# Autodesk Inventor assembly: eMachineShop.20
(part 2 of 2)
- D:\Tesis\Modelo 3D\CAD\Electronicos\MC15A_V5\MC15A_V5_1779569544.214\MC15A_V5_1779569544.214\eMachineShop.20.315.ipt
- D:\Tesis\Modelo 3D\CAD\Electronicos\MC15A_V5\MC15A_V5_1779569544.214\MC15A_V5_1779569544.214\eMachineShop.20.316.ipt
- D:\Tesis\Modelo 3D\CAD\Electronicos\MC15A_V5\MC15A_V5_1779569544.214\MC15A_V5_1779569544.214\eMachineShop.20.317.ipt
- D:\Tesis\Modelo 3D\CAD\Electronicos\MC15A_V5\MC15A_V5_1779569544.214\MC15A_V5_1779569544.214\eMachineShop.20.318.ipt
- D:\Tesis\Modelo 3D\CAD\Electronicos\MC15A_V5\MC15A_V5_1779569544.214\MC15A_V5_1779569544.214\eMachineShop.20.319.ipt
- D:\Tesis\Modelo 3D\CAD\Electronicos\MC15A_V5\MC15A_V5_1779569544.214\MC15A_V5_1779569544.214\eMachineShop.20.320.ipt
- D:\Tesis\Modelo 3D\CAD\Electronicos\MC15A_V5\MC15A_V5_1779569544.214\MC15A_V5_1779569544.214\eMachineShop.20.321.ipt
- D:\Tesis\Modelo 3D\CAD\Electronicos\MC15A_V5\MC15A_V5_1779569544.214\MC15A_V5_1779569544.214\eMachineShop.20.322.ipt
- D:\Tesis\Modelo 3D\CAD\Electronicos\MC15A_V5\MC15A_V5_1779569544.214\MC15A_V5_1779569544.214\eMachineShop.20.323.ipt
- D:\Tesis\Modelo 3D\CAD\Electronicos\MC15A_V5\MC15A_V5_1779569544.214\MC15A_V5_1779569544.214\eMachineShop.20.324.ipt
- D:\Tesis\Modelo 3D\CAD\Electronicos\MC15A_V5\MC15A_V5_1779569544.214\MC15A_V5_1779569544.214\eMachineShop.20.325.ipt
- D:\Tesis\Modelo 3D\CAD\Electronicos\MC15A_V5\MC15A_V5_1779569544.214\MC15A_V5_1779569544.214\eMachineShop.20.326.ipt
- D:\Tesis\Modelo 3D\CAD\Electronicos\MC15A_V5\MC15A_V5_1779569544.214\MC15A_V5_1779569544.214\eMachineShop.20.327.ipt
- D:\Tesis\Modelo 3D\CAD\Electronicos\MC15A_V5\MC15A_V5_1779569544.214\MC15A_V5_1779569544.214\eMachineShop.20.328.ipt
- D:\Tesis\Modelo 3D\CAD\Electronicos\MC15A_V5\MC15A_V5_1779569544.214\MC15A_V5_1779569544.214\eMachineShop.20.329.ipt
- D:\Tesis\Modelo 3D\CAD\Electronicos\MC15A_V5\MC15A_V5_1779569544.214\MC15A_V5_1779569544.214\eMachineShop.20.330.ipt
- D:\Tesis\Modelo 3D\CAD\Electronicos\MC15A_V5\MC15A_V5_1779569544.214\MC15A_V5_1779569544.214\eMachineShop.20.331.ipt
- D:\Tesis\Modelo 3D\CAD\Electronicos\MC15A_V5\MC15A_V5_1779569544.214\MC15A_V5_1779569544.214\eMachineShop.20.332.ipt
- D:\Tesis\Modelo 3D\CAD\Electronicos\MC15A_V5\MC15A_V5_1779569544.214\MC15A_V5_1779569544.214\eMachineShop.20.333.ipt
- D:\Tesis\Modelo 3D\CAD\Electronicos\MC15A_V5\MC15A_V5_1779569544.214\MC15A_V5_1779569544.214\eMachineShop.20.334.ipt
- D:\Tesis\Modelo 3D\CAD\Electronicos\MC15A_V5\MC15A_V5_1779569544.214\MC15A_V5_1779569544.214\eMachineShop.20.335.ipt
- D:\Tesis\Modelo 3D\CAD\Electronicos\MC15A_V5\MC15A_V5_1779569544.214\MC15A_V5_1779569544.214\eMachineShop.20.336.ipt
- D:\Tesis\Modelo 3D\CAD\Electronicos\MC15A_V5\MC15A_V5_1779569544.214\MC15A_V5_1779569544.214\eMachineShop.20.337.ipt
- D:\Tesis\Modelo 3D\CAD\Electronicos\MC15A_V5\MC15A_V5_1779569544.214\MC15A_V5_1779569544.214\eMachineShop.20.338.ipt
- D:\Tesis\Modelo 3D\CAD\Electronicos\MC15A_V5\MC15A_V5_1779569544.214\MC15A_V5_1779569544.214\eMachineShop.20.339.ipt
- D:\Tesis\Modelo 3D\CAD\Electronicos\MC15A_V5\MC15A_V5_1779569544.214\MC15A_V5_1779569544.214\eMachineShop.20.340.ipt
- D:\Tesis\Modelo 3D\CAD\Electronicos\MC15A_V5\MC15A_V5_1779569544.214\MC15A_V5_1779569544.214\eMachineShop.20.341.ipt
- D:\Tesis\Modelo 3D\CAD\Electronicos\MC15A_V5\MC15A_V5_1779569544.214\MC15A_V5_1779569544.214\eMachineShop.20.342.ipt
- D:\Tesis\Modelo 3D\CAD\Electronicos\MC15A_V5\MC15A_V5_1779569544.214\MC15A_V5_1779569544.214\eMachineShop.20.343.ipt
- D:\Tesis\Modelo 3D\CAD\Electronicos\MC15A_V5\MC15A_V5_1779569544.214\MC15A_V5_1779569544.214\eMachineShop.20.344.ipt
- D:\Tesis\Modelo 3D\CAD\Electronicos\MC15A_V5\MC15A_V5_1779569544.214\MC15A_V5_1779569544.214\eMachineShop.20.345.ipt
- D:\Tesis\Modelo 3D\CAD\Electronicos\MC15A_V5\MC15A_V5_1779569544.214\MC15A_V5_1779569544.214\eMachineShop.20.346.ipt
- D:\Tesis\Modelo 3D\CAD\Electronicos\MC15A_V5\MC15A_V5_1779569544.214\MC15A_V5_1779569544.214\eMachineShop.20.347.ipt
- D:\Tesis\Modelo 3D\CAD\Electronicos\MC15A_V5\MC15A_V5_1779569544.214\MC15A_V5_1779569544.214\eMachineShop.20.348.ipt
- D:\Tesis\Modelo 3D\CAD\Electronicos\MC15A_V5\MC15A_V5_1779569544.214\MC15A_V5_1779569544.214\eMachineShop.20.349.ipt
- D:\Tesis\Modelo 3D\CAD\Electronicos\MC15A_V5\MC15A_V5_1779569544.214\MC15A_V5_1779569544.214\eMachineShop.20.350.ipt
- D:\Tesis\Modelo 3D\CAD\Electronicos\MC15A_V5\MC15A_V5_1779569544.214\MC15A_V5_1779569544.214\eMachineShop.20.351.ipt
- D:\Tesis\Modelo 3D\CAD\Electronicos\MC15A_V5\MC15A_V5_1779569544.214\MC15A_V5_1779569544.214\eMachineShop.20.352.ipt
- D:\Tesis\Modelo 3D\CAD\Electronicos\MC15A_V5\MC15A_V5_1779569544.214\MC15A_V5_1779569544.214\eMachineShop.20.353.ipt
- D:\Tesis\Modelo 3D\CAD\Electronicos\MC15A_V5\MC15A_V5_1779569544.214\MC15A_V5_1779569544.214\eMachineShop.20.354.ipt
- D:\Tesis\Modelo 3D\CAD\Electronicos\MC15A_V5\MC15A_V5_1779569544.214\MC15A_V5_1779569544.214\eMachineShop.20.355.ipt
- D:\Tesis\Modelo 3D\CAD\Electronicos\MC15A_V5\MC15A_V5_1779569544.214\MC15A_V5_1779569544.214\eMachineShop.20.356.ipt
- D:\Tesis\Modelo 3D\CAD\Electronicos\MC15A_V5\MC15A_V5_1779569544.214\MC15A_V5_1779569544.214\eMachineShop.20.357.ipt
- D:\Tesis\Modelo 3D\CAD\Electronicos\MC15A_V5\MC15A_V5_1779569544.214\MC15A_V5_1779569544.214\eMachineShop.20.358.ipt
- D:\Tesis\Modelo 3D\CAD\Electronicos\MC15A_V5\MC15A_V5_1779569544.214\MC15A_V5_1779569544.214\eMachineShop.20.359.ipt
- D:\Tesis\Modelo 3D\CAD\Electronicos\MC15A_V5\MC15A_V5_1779569544.214\MC15A_V5_1779569544.214\eMachineShop.20.360.ipt
- D:\Tesis\Modelo 3D\CAD\Electronicos\MC15A_V5\MC15A_V5_1779569544.214\MC15A_V5_1779569544.214\eMachineShop.20.361.ipt
- D:\Tesis\Modelo 3D\CAD\Electronicos\MC15A_V5\MC15A_V5_1779569544.214\MC15A_V5_1779569544.214\eMachineShop.20.362.ipt
- D:\Tesis\Modelo 3D\CAD\Electronicos\MC15A_V5\MC15A_V5_1779569544.214\MC15A_V5_1779569544.214\eMachineShop.20.363.ipt
- D:\Tesis\Modelo 3D\CAD\Electronicos\MC15A_V5\MC15A_V5_1779569544.214\MC15A_V5_1779569544.214\eMachineShop.20.364.ipt
- D:\Tesis\Modelo 3D\CAD\Electronicos\MC15A_V5\MC15A_V5_1779569544.214\MC15A_V5_1779569544.214\eMachineShop.20.365.ipt
- D:\Tesis\Modelo 3D\CAD\Electronicos\MC15A_V5\MC15A_V5_1779569544.214\MC15A_V5_1779569544.214\eMachineShop.20.366.ipt
- D:\Tesis\Modelo 3D\CAD\Electronicos\MC15A_V5\MC15A_V5_1779569544.214\MC15A_V5_1779569544.214\eMachineShop.20.367.ipt
- D:\Tesis\Modelo 3D\CAD\Electronicos\MC15A_V5\MC15A_V5_1779569544.214\MC15A_V5_1779569544.214\eMachineShop.20.368.ipt
- D:\Tesis\Modelo 3D\CAD\Electronicos\MC15A_V5\MC15A_V5_1779569544.214\MC15A_V5_1779569544.214\eMachineShop.20.369.ipt
- D:\Tesis\Modelo 3D\CAD\Electronicos\MC15A_V5\MC15A_V5_1779569544.214\MC15A_V5_1779569544.214\eMachineShop.20.370.ipt
- D:\Tesis\Modelo 3D\CAD\Electronicos\MC15A_V5\MC15A_V5_1779569544.214\MC15A_V5_1779569544.214\eMachineShop.20.371.ipt
- D:\Tesis\Modelo 3D\CAD\Electronicos\MC15A_V5\MC15A_V5_1779569544.214\MC15A_V5_1779569544.214\eMachineShop.20.372.ipt
- D:\Tesis\Modelo 3D\CAD\Electronicos\MC15A_V5\MC15A_V5_1779569544.214\MC15A_V5_1779569544.214\eMachineShop.20.373.ipt
- D:\Tesis\Modelo 3D\CAD\Electronicos\MC15A_V5\MC15A_V5_1779569544.214\MC15A_V5_1779569544.214\eMachineShop.20.374.ipt
- D:\Tesis\Modelo 3D\CAD\Electronicos\MC15A_V5\MC15A_V5_1779569544.214\MC15A_V5_1779569544.214\eMachineShop.20.375.ipt
- D:\Tesis\Modelo 3D\CAD\Electronicos\MC15A_V5\MC15A_V5_1779569544.214\MC15A_V5_1779569544.214\eMachineShop.20.376.ipt
- D:\Tesis\Modelo 3D\CAD\Electronicos\MC15A_V5\MC15A_V5_1779569544.214\MC15A_V5_1779569544.214\eMachineShop.20.377.ipt
- D:\Tesis\Modelo 3D\CAD\Electronicos\MC15A_V5\MC15A_V5_1779569544.214\MC15A_V5_1779569544.214\eMachineShop.20.378.ipt
- D:\Tesis\Modelo 3D\CAD\Electronicos\MC15A_V5\MC15A_V5_1779569544.214\MC15A_V5_1779569544.214\eMachineShop.20.379.ipt
- D:\Tesis\Modelo 3D\CAD\Electronicos\MC15A_V5\MC15A_V5_1779569544.214\MC15A_V5_1779569544.214\eMachineShop.20.380.ipt
- D:\Tesis\Modelo 3D\CAD\Electronicos\MC15A_V5\MC15A_V5_1779569544.214\MC15A_V5_1779569544.214\eMachineShop.20.381.ipt
- D:\Tesis\Modelo 3D\CAD\Electronicos\MC15A_V5\MC15A_V5_1779569544.214\MC15A_V5_1779569544.214\eMachineShop.20.382.ipt
- D:\Tesis\Modelo 3D\CAD\Electronicos\MC15A_V5\MC15A_V5_1779569544.214\MC15A_V5_1779569544.214\eMachineShop.20.383.ipt
- D:\Tesis\Modelo 3D\CAD\Electronicos\MC15A_V5\MC15A_V5_1779569544.214\MC15A_V5_1779569544.214\eMachineShop.20.384.ipt
- D:\Tesis\Modelo 3D\CAD\Electronicos\MC15A_V5\MC15A_V5_1779569544.214\MC15A_V5_1779569544.214\eMachineShop.20.385.ipt
- D:\Tesis\Modelo 3D\CAD\Electronicos\MC15A_V5\MC15A_V5_1779569544.214\MC15A_V5_1779569544.214\eMachineShop.20.386.ipt
- D:\Tesis\Modelo 3D\CAD\Electronicos\MC15A_V5\MC15A_V5_1779569544.214\MC15A_V5_1779569544.214\eMachineShop.20.387.ipt
- D:\Tesis\Modelo 3D\CAD\Electronicos\MC15A_V5\MC15A_V5_1779569544.214\MC15A_V5_1779569544.214\eMachineShop.20.388.ipt
- D:\Tesis\Modelo 3D\CAD\Electronicos\MC15A_V5\MC15A_V5_1779569544.214\MC15A_V5_1779569544.214\eMachineShop.20.389.ipt
- D:\Tesis\Modelo 3D\CAD\Electronicos\MC15A_V5\MC15A_V5_1779569544.214\MC15A_V5_1779569544.214\eMachineShop.20.390.ipt
- D:\Tesis\Modelo 3D\CAD\Electronicos\MC15A_V5\MC15A_V5_1779569544.214\MC15A_V5_1779569544.214\eMachineShop.20.391.ipt
- D:\Tesis\Modelo 3D\CAD\Electronicos\MC15A_V5\MC15A_V5_1779569544.214\MC15A_V5_1779569544.214\eMachineShop.20.392.ipt
- D:\Tesis\Modelo 3D\CAD\Electronicos\MC15A_V5\MC15A_V5_1779569544.214\MC15A_V5_1779569544.214\eMachineShop.20.393.ipt
- D:\Tesis\Modelo 3D\CAD\Electronicos\MC15A_V5\MC15A_V5_1779569544.214\MC15A_V5_1779569544.214\eMachineShop.20.394.ipt
- D:\Tesis\Modelo 3D\CAD\Electronicos\MC15A_V5\MC15A_V5_1779569544.214\MC15A_V5_1779569544.214\eMachineShop.20.395.ipt
- D:\Tesis\Modelo 3D\CAD\Electronicos\MC15A_V5\MC15A_V5_1779569544.214\MC15A_V5_1779569544.214\eMachineShop.20.396.ipt
- D:\Tesis\Modelo 3D\CAD\Electronicos\MC15A_V5\MC15A_V5_1779569544.214\MC15A_V5_1779569544.214\eMachineShop.20.397.ipt
- D:\Tesis\Modelo 3D\CAD\Electronicos\MC15A_V5\MC15A_V5_1779569544.214\MC15A_V5_1779569544.214\eMachineShop.20.398.ipt
- D:\Tesis\Modelo 3D\CAD\Electronicos\MC15A_V5\MC15A_V5_1779569544.214\MC15A_V5_1779569544.214\eMachineShop.20.399.ipt
- D:\Tesis\Modelo 3D\CAD\Electronicos\MC15A_V5\MC15A_V5_1779569544.214\MC15A_V5_1779569544.214\eMachineShop.20.400.ipt
- D:\Tesis\Modelo 3D\CAD\Electronicos\MC15A_V5\MC15A_V5_1779569544.214\MC15A_V5_1779569544.214\eMachineShop.20.401.ipt
- D:\Tesis\Modelo 3D\CAD\Electronicos\MC15A_V5\MC15A_V5_1779569544.214\MC15A_V5_1779569544.214\eMachineShop.20.402.ipt
- D:\Tesis\Modelo 3D\CAD\Electronicos\MC15A_V5\MC15A_V5_1779569544.214\MC15A_V5_1779569544.214\eMachineShop.20.403.ipt
- D:\Tesis\Modelo 3D\CAD\Electronicos\MC15A_V5\MC15A_V5_1779569544.214\MC15A_V5_1779569544.214\eMachineShop.20.404.ipt
- D:\Tesis\Modelo 3D\CAD\Electronicos\MC15A_V5\MC15A_V5_1779569544.214\MC15A_V5_1779569544.214\eMachineShop.20.405.ipt
- D:\Tesis\Modelo 3D\CAD\Electronicos\MC15A_V5\MC15A_V5_1779569544.214\MC15A_V5_1779569544.214\eMachineShop.20.406.ipt
- D:\Tesis\Modelo 3D\CAD\Electronicos\MC15A_V5\MC15A_V5_1779569544.214\MC15A_V5_1779569544.214\eMachineShop.20.407.ipt
- D:\Tesis\Modelo 3D\CAD\Electronicos\MC15A_V5\MC15A_V5_1779569544.214\MC15A_V5_1779569544.214\eMachineShop.20.408.ipt
- D:\Tesis\Modelo 3D\CAD\Electronicos\MC15A_V5\MC15A_V5_1779569544.214\MC15A_V5_1779569544.214\eMachineShop.20.409.ipt
- D:\Tesis\Modelo 3D\CAD\Electronicos\MC15A_V5\MC15A_V5_1779569544.214\MC15A_V5_1779569544.214\eMachineShop.20.410.ipt
- D:\Tesis\Modelo 3D\CAD\Electronicos\MC15A_V5\MC15A_V5_1779569544.214\MC15A_V5_1779569544.214\eMachineShop.20.411.ipt
- D:\Tesis\Modelo 3D\CAD\Electronicos\MC15A_V5\MC15A_V5_1779569544.214\MC15A_V5_1779569544.214\eMachineShop.20.412.ipt
- D:\Tesis\Modelo 3D\CAD\Electronicos\MC15A_V5\MC15A_V5_1779569544.214\MC15A_V5_1779569544.214\eMachineShop.20.413.ipt
- D:\Tesis\Modelo 3D\CAD\Electronicos\MC15A_V5\MC15A_V5_1779569544.214\MC15A_V5_1779569544.214\eMachineShop.20.414.ipt
- D:\Tesis\Modelo 3D\CAD\Electronicos\MC15A_V5\MC15A_V5_1779569544.214\MC15A_V5_1779569544.214\eMachineShop.20.415.ipt
- D:\Tesis\Modelo 3D\CAD\Electronicos\MC15A_V5\MC15A_V5_1779569544.214\MC15A_V5_1779569544.214\eMachineShop.20.416.ipt
- D:\Tesis\Modelo 3D\CAD\Electronicos\MC15A_V5\MC15A_V5_1779569544.214\MC15A_V5_1779569544.214\eMachineShop.20.417.ipt
- D:\Tesis\Modelo 3D\CAD\Electronicos\MC15A_V5\MC15A_V5_1779569544.214\MC15A_V5_1779569544.214\eMachineShop.20.418.ipt
- D:\Tesis\Modelo 3D\CAD\Electronicos\MC15A_V5\MC15A_V5_1779569544.214\MC15A_V5_1779569544.214\eMachineShop.20.419.ipt
- D:\Tesis\Modelo 3D\CAD\Electronicos\MC15A_V5\MC15A_V5_1779569544.214\MC15A_V5_1779569544.214\eMachineShop.20.420.ipt
- D:\Tesis\Modelo 3D\CAD\Electronicos\MC15A_V5\MC15A_V5_1779569544.214\MC15A_V5_1779569544.214\eMachineShop.20.421.ipt
- D:\Tesis\Modelo 3D\CAD\Electronicos\MC15A_V5\MC15A_V5_1779569544.214\MC15A_V5_1779569544.214\eMachineShop.20.422.ipt
- D:\Tesis\Modelo 3D\CAD\Electronicos\MC15A_V5\MC15A_V5_1779569544.214\MC15A_V5_1779569544.214\eMachineShop.20.423.ipt
- D:\Tesis\Modelo 3D\CAD\Electronicos\MC15A_V5\MC15A_V5_1779569544.214\MC15A_V5_1779569544.214\eMachineShop.20.424.ipt
- D:\Tesis\Modelo 3D\CAD\Electronicos\MC15A_V5\MC15A_V5_1779569544.214\MC15A_V5_1779569544.214\eMachineShop.20.425.ipt
- D:\Tesis\Modelo 3D\CAD\Electronicos\MC15A_V5\MC15A_V5_1779569544.214\MC15A_V5_1779569544.214\eMachineShop.20.426.ipt
- D:\Tesis\Modelo 3D\CAD\Electronicos\MC15A_V5\MC15A_V5_1779569544.214\MC15A_V5_1779569544.214\eMachineShop.20.427.ipt
- D:\Tesis\Modelo 3D\CAD\Electronicos\MC15A_V5\MC15A_V5_1779569544.214\MC15A_V5_1779569544.214\eMachineShop.20.428.ipt
- D:\Tesis\Modelo 3D\CAD\Electronicos\MC15A_V5\MC15A_V5_1779569544.214\MC15A_V5_1779569544.214\eMachineShop.20.429.ipt
- D:\Tesis\Modelo 3D\CAD\Electronicos\MC15A_V5\MC15A_V5_1779569544.214\MC15A_V5_1779569544.214\eMachineShop.20.430.ipt
- D:\Tesis\Modelo 3D\CAD\Electronicos\MC15A_V5\MC15A_V5_1779569544.214\MC15A_V5_1779569544.214\eMachineShop.20.431.ipt
- D:\Tesis\Modelo 3D\CAD\Electronicos\MC15A_V5\MC15A_V5_1779569544.214\MC15A_V5_1779569544.214\eMachineShop.20.432.ipt
- D:\Tesis\Modelo 3D\CAD\Electronicos\MC15A_V5\MC15A_V5_1779569544.214\MC15A_V5_1779569544.214\eMachineShop.20.433.ipt
- D:\Tesis\Modelo 3D\CAD\Electronicos\MC15A_V5\MC15A_V5_1779569544.214\MC15A_V5_1779569544.214\eMachineShop.20.434.ipt
- D:\Tesis\Modelo 3D\CAD\Electronicos\MC15A_V5\MC15A_V5_1779569544.214\MC15A_V5_1779569544.214\eMachineShop.20.435.ipt
- D:\Tesis\Modelo 3D\CAD\Electronicos\MC15A_V5\MC15A_V5_1779569544.214\MC15A_V5_1779569544.214\eMachineShop.20.436.ipt
- D:\Tesis\Modelo 3D\CAD\Electronicos\MC15A_V5\MC15A_V5_1779569544.214\MC15A_V5_1779569544.214\eMachineShop.20.437.ipt
- D:\Tesis\Modelo 3D\CAD\Electronicos\MC15A_V5\MC15A_V5_1779569544.214\MC15A_V5_1779569544.214\eMachineShop.20.438.ipt
- D:\Tesis\Modelo 3D\CAD\Electronicos\MC15A_V5\MC15A_V5_1779569544.214\MC15A_V5_1779569544.214\eMachineShop.20.439.ipt
- D:\Tesis\Modelo 3D\CAD\Electronicos\MC15A_V5\MC15A_V5_1779569544.214\MC15A_V5_1779569544.214\eMachineShop.20.440.ipt
- D:\Tesis\Modelo 3D\CAD\Electronicos\MC15A_V5\MC15A_V5_1779569544.214\MC15A_V5_1779569544.214\eMachineShop.20.441.ipt
- D:\Tesis\Modelo 3D\CAD\Electronicos\MC15A_V5\MC15A_V5_1779569544.214\MC15A_V5_1779569544.214\eMachineShop.20.442.ipt
- D:\Tesis\Modelo 3D\CAD\Electronicos\MC15A_V5\MC15A_V5_1779569544.214\MC15A_V5_1779569544.214\eMachineShop.20.443.ipt
- D:\Tesis\Modelo 3D\CAD\Electronicos\MC15A_V5\MC15A_V5_1779569544.214\MC15A_V5_1779569544.214\eMachineShop.20.444.ipt
- D:\Tesis\Modelo 3D\CAD\Electronicos\MC15A_V5\MC15A_V5_1779569544.214\MC15A_V5_1779569544.214\eMachineShop.20.445.ipt
- D:\Tesis\Modelo 3D\CAD\Electronicos\MC15A_V5\MC15A_V5_1779569544.214\MC15A_V5_1779569544.214\eMachineShop.20.446.ipt
- D:\Tesis\Modelo 3D\CAD\Electronicos\MC15A_V5\MC15A_V5_1779569544.214\MC15A_V5_1779569544.214\eMachineShop.20.447.ipt
- D:\Tesis\Modelo 3D\CAD\Electronicos\MC15A_V5\MC15A_V5_1779569544.214\MC15A_V5_1779569544.214\eMachineShop.20.448.ipt
- D:\Tesis\Modelo 3D\CAD\Electronicos\MC15A_V5\MC15A_V5_1779569544.214\MC15A_V5_1779569544.214\eMachineShop.20.449.ipt
- D:\Tesis\Modelo 3D\CAD\Electronicos\MC15A_V5\MC15A_V5_1779569544.214\MC15A_V5_1779569544.214\eMachineShop.20.450.ipt
- D:\Tesis\Modelo 3D\CAD\Electronicos\MC15A_V5\MC15A_V5_1779569544.214\MC15A_V5_1779569544.214\eMachineShop.20.451.ipt
- D:\Tesis\Modelo 3D\CAD\Electronicos\MC15A_V5\MC15A_V5_1779569544.214\MC15A_V5_1779569544.214\eMachineShop.20.452.ipt
- D:\Tesis\Modelo 3D\CAD\Electronicos\MC15A_V5\MC15A_V5_1779569544.214\MC15A_V5_1779569544.214\eMachineShop.20.453.ipt
- D:\Tesis\Modelo 3D\CAD\Electronicos\MC15A_V5\MC15A_V5_1779569544.214\MC15A_V5_1779569544.214\eMachineShop.20.454.ipt
- D:\Tesis\Modelo 3D\CAD\Electronicos\MC15A_V5\MC15A_V5_1779569544.214\MC15A_V5_1779569544.214\eMachineShop.20.455.ipt
- D:\Tesis\Modelo 3D\CAD\Electronicos\MC15A_V5\MC15A_V5_1779569544.214\MC15A_V5_1779569544.214\eMachineShop.20.456.ipt
- D:\Tesis\Modelo 3D\CAD\Electronicos\MC15A_V5\MC15A_V5_1779569544.214\MC15A_V5_1779569544.214\eMachineShop.20.457.ipt
- D:\Tesis\Modelo 3D\CAD\Electronicos\MC15A_V5\MC15A_V5_1779569544.214\MC15A_V5_1779569544.214\eMachineShop.20.458.ipt
- D:\Tesis\Modelo 3D\CAD\Electronicos\MC15A_V5\MC15A_V5_1779569544.214\MC15A_V5_1779569544.214\eMachineShop.20.459.ipt
- D:\Tesis\Modelo 3D\CAD\Electronicos\MC15A_V5\MC15A_V5_1779569544.214\MC15A_V5_1779569544.214\eMachineShop.20.460.ipt
- D:\Tesis\Modelo 3D\CAD\Electronicos\MC15A_V5\MC15A_V5_1779569544.214\MC15A_V5_1779569544.214\eMachineShop.20.461.ipt
- D:\Tesis\Modelo 3D\CAD\Electronicos\MC15A_V5\MC15A_V5_1779569544.214\MC15A_V5_1779569544.214\eMachineShop.20.462.ipt
- D:\Tesis\Modelo 3D\CAD\Electronicos\MC15A_V5\MC15A_V5_1779569544.214\MC15A_V5_1779569544.214\eMachineShop.20.463.ipt
- D:\Tesis\Modelo 3D\CAD\Electronicos\MC15A_V5\MC15A_V5_1779569544.214\MC15A_V5_1779569544.214\eMachineShop.20.464.ipt
- D:\Tesis\Modelo 3D\CAD\Electronicos\MC15A_V5\MC15A_V5_1779569544.214\MC15A_V5_1779569544.214\eMachineShop.20.465.ipt
- D:\Tesis\Modelo 3D\CAD\Electronicos\MC15A_V5\MC15A_V5_1779569544.214\MC15A_V5_1779569544.214\eMachineShop.20.466.ipt
- D:\Tesis\Modelo 3D\CAD\Electronicos\MC15A_V5\MC15A_V5_1779569544.214\MC15A_V5_1779569544.214\eMachineShop.20.467.ipt
- D:\Tesis\Modelo 3D\CAD\Electronicos\MC15A_V5\MC15A_V5_1779569544.214\MC15A_V5_1779569544.214\eMachineShop.20.468.ipt
- D:\Tesis\Modelo 3D\CAD\Electronicos\MC15A_V5\MC15A_V5_1779569544.214\MC15A_V5_1779569544.214\eMachineShop.20.469.ipt
- D:\Tesis\Modelo 3D\CAD\Electronicos\MC15A_V5\MC15A_V5_1779569544.214\MC15A_V5_1779569544.214\eMachineShop.20.470.ipt
- D:\Tesis\Modelo 3D\CAD\Electronicos\MC15A_V5\MC15A_V5_1779569544.214\MC15A_V5_1779569544.214\eMachineShop.20.471.ipt
- D:\Tesis\Modelo 3D\CAD\Electronicos\MC15A_V5\MC15A_V5_1779569544.214\MC15A_V5_1779569544.214\eMachineShop.20.472.ipt
- D:\Tesis\Modelo 3D\CAD\Electronicos\MC15A_V5\MC15A_V5_1779569544.214\MC15A_V5_1779569544.214\eMachineShop.20.473.ipt
- D:\Tesis\Modelo 3D\CAD\Electronicos\MC15A_V5\MC15A_V5_1779569544.214\MC15A_V5_1779569544.214\eMachineShop.20.474.ipt
- D:\Tesis\Modelo 3D\CAD\Electronicos\MC15A_V5\MC15A_V5_1779569544.214\MC15A_V5_1779569544.214\eMachineShop.20.475.ipt
- D:\Tesis\Modelo 3D\CAD\Electronicos\MC15A_V5\MC15A_V5_1779569544.214\MC15A_V5_1779569544.214\eMachineShop.20.476.ipt
- D:\Tesis\Modelo 3D\CAD\Electronicos\MC15A_V5\MC15A_V5_1779569544.214\MC15A_V5_1779569544.214\eMachineShop.20.477.ipt
- D:\Tesis\Modelo 3D\CAD\Electronicos\MC15A_V5\MC15A_V5_1779569544.214\MC15A_V5_1779569544.214\eMachineShop.20.478.ipt
- D:\Tesis\Modelo 3D\CAD\Electronicos\MC15A_V5\MC15A_V5_1779569544.214\MC15A_V5_1779569544.214\eMachineShop.20.479.ipt
- D:\Tesis\Modelo 3D\CAD\Electronicos\MC15A_V5\MC15A_V5_1779569544.214\MC15A_V5_1779569544.214\eMachineShop.20.480.ipt
- D:\Tesis\Modelo 3D\CAD\Electronicos\MC15A_V5\MC15A_V5_1779569544.214\MC15A_V5_1779569544.214\eMachineShop.20.481.ipt
- D:\Tesis\Modelo 3D\CAD\Electronicos\MC15A_V5\MC15A_V5_1779569544.214\MC15A_V5_1779569544.214\eMachineShop.20.482.ipt
- D:\Tesis\Modelo 3D\CAD\Electronicos\MC15A_V5\MC15A_V5_1779569544.214\MC15A_V5_1779569544.214\eMachineShop.20.483.ipt
- D:\Tesis\Modelo 3D\CAD\Electronicos\MC15A_V5\MC15A_V5_1779569544.214\MC15A_V5_1779569544.214\eMachineShop.20.484.ipt
- D:\Tesis\Modelo 3D\CAD\Electronicos\MC15A_V5\MC15A_V5_1779569544.214\MC15A_V5_1779569544.214\eMachineShop.20.485.ipt
- D:\Tesis\Modelo 3D\CAD\Electronicos\MC15A_V5\MC15A_V5_1779569544.214\MC15A_V5_1779569544.214\eMachineShop.20.486.ipt
- D:\Tesis\Modelo 3D\CAD\Electronicos\MC15A_V5\MC15A_V5_1779569544.214\MC15A_V5_1779569544.214\eMachineShop.20.487.ipt
- D:\Tesis\Modelo 3D\CAD\Electronicos\MC15A_V5\MC15A_V5_1779569544.214\MC15A_V5_1779569544.214\eMachineShop.20.488.ipt
- D:\Tesis\Modelo 3D\CAD\Electronicos\MC15A_V5\MC15A_V5_1779569544.214\MC15A_V5_1779569544.214\eMachineShop.20.489.ipt
- D:\Tesis\Modelo 3D\CAD\Electronicos\MC15A_V5\MC15A_V5_1779569544.214\MC15A_V5_1779569544.214\eMachineShop.20.490.ipt
- D:\Tesis\Modelo 3D\CAD\Electronicos\MC15A_V5\MC15A_V5_1779569544.214\MC15A_V5_1779569544.214\eMachineShop.20.491.ipt
- D:\Tesis\Modelo 3D\CAD\Electronicos\MC15A_V5\MC15A_V5_1779569544.214\MC15A_V5_1779569544.214\eMachineShop.20.492.ipt
- D:\Tesis\Modelo 3D\CAD\Electronicos\MC15A_V5\MC15A_V5_1779569544.214\MC15A_V5_1779569544.214\eMachineShop.20.493.ipt
- D:\Tesis\Modelo 3D\CAD\Electronicos\MC15A_V5\MC15A_V5_1779569544.214\MC15A_V5_1779569544.214\eMachineShop.20.494.ipt
- D:\Tesis\Modelo 3D\CAD\Electronicos\MC15A_V5\MC15A_V5_1779569544.214\MC15A_V5_1779569544.214\eMachineShop.20.495.ipt
- D:\Tesis\Modelo 3D\CAD\Electronicos\MC15A_V5\MC15A_V5_1779569544.214\MC15A_V5_1779569544.214\eMachineShop.20.496.ipt
- D:\Tesis\Modelo 3D\CAD\Electronicos\MC15A_V5\MC15A_V5_1779569544.214\MC15A_V5_1779569544.214\eMachineShop.20.497.ipt
- D:\Tesis\Modelo 3D\CAD\Electronicos\MC15A_V5\MC15A_V5_1779569544.214\MC15A_V5_1779569544.214\eMachineShop.20.498.ipt
- D:\Tesis\Modelo 3D\CAD\Electronicos\MC15A_V5\MC15A_V5_1779569544.214\MC15A_V5_1779569544.214\eMachineShop.20.499.ipt
- D:\Tesis\Modelo 3D\CAD\Electronicos\MC15A_V5\MC15A_V5_1779569544.214\MC15A_V5_1779569544.214\eMachineShop.20.500.ipt
- D:\Tesis\Modelo 3D\CAD\Electronicos\MC15A_V5\MC15A_V5_1779569544.214\MC15A_V5_1779569544.214\eMachineShop.20.501.ipt
- D:\Tesis\Modelo 3D\CAD\Electronicos\MC15A_V5\MC15A_V5_1779569544.214\MC15A_V5_1779569544.214\eMachineShop.20.502.ipt
- D:\Tesis\Modelo 3D\CAD\Electronicos\MC15A_V5\MC15A_V5_1779569544.214\MC15A_V5_1779569544.214\eMachineShop.20.503.ipt
- D:\Tesis\Modelo 3D\CAD\Electronicos\MC15A_V5\MC15A_V5_1779569544.214\MC15A_V5_1779569544.214\eMachineShop.20.504.ipt
- D:\Tesis\Modelo 3D\CAD\Electronicos\MC15A_V5\MC15A_V5_1779569544.214\MC15A_V5_1779569544.214\eMachineShop.20.505.ipt
- D:\Tesis\Modelo 3D\CAD\Electronicos\MC15A_V5\MC15A_V5_1779569544.214\MC15A_V5_1779569544.214\eMachineShop.20.506.ipt
- D:\Tesis\Modelo 3D\CAD\Electronicos\MC15A_V5\MC15A_V5_1779569544.214\MC15A_V5_1779569544.214\eMachineShop.20.507.ipt
- D:\Tesis\Modelo 3D\CAD\Electronicos\MC15A_V5\MC15A_V5_1779569544.214\MC15A_V5_1779569544.214\eMachineShop.20.508.ipt
- D:\Tesis\Modelo 3D\CAD\Electronicos\MC15A_V5\MC15A_V5_1779569544.214\MC15A_V5_1779569544.214\eMachineShop.20.509.ipt
- D:\Tesis\Modelo 3D\CAD\Electronicos\MC15A_V5\MC15A_V5_1779569544.214\MC15A_V5_1779569544.214\eMachineShop.20.510.ipt
- D:\Tesis\Modelo 3D\CAD\Electronicos\MC15A_V5\MC15A_V5_1779569544.214\MC15A_V5_1779569544.214\eMachineShop.20.511.ipt
- D:\Tesis\Modelo 3D\CAD\Electronicos\MC15A_V5\MC15A_V5_1779569544.214\MC15A_V5_1779569544.214\eMachineShop.20.512.ipt
- D:\Tesis\Modelo 3D\CAD\Electronicos\MC15A_V5\MC15A_V5_1779569544.214\MC15A_V5_1779569544.214\eMachineShop.20.513.ipt
- D:\Tesis\Modelo 3D\CAD\Electronicos\MC15A_V5\MC15A_V5_1779569544.214\MC15A_V5_1779569544.214\eMachineShop.20.514.ipt
- D:\Tesis\Modelo 3D\CAD\Electronicos\MC15A_V5\MC15A_V5_1779569544.214\MC15A_V5_1779569544.214\eMachineShop.20.515.ipt
- D:\Tesis\Modelo 3D\CAD\Electronicos\MC15A_V5\MC15A_V5_1779569544.214\MC15A_V5_1779569544.214\eMachineShop.20.516.ipt
- D:\Tesis\Modelo 3D\CAD\Electronicos\MC15A_V5\MC15A_V5_1779569544.214\MC15A_V5_1779569544.214\eMachineShop.20.517.ipt
- D:\Tesis\Modelo 3D\CAD\Electronicos\MC15A_V5\MC15A_V5_1779569544.214\MC15A_V5_1779569544.214\eMachineShop.20.518.ipt
- D:\Tesis\Modelo 3D\CAD\Electronicos\MC15A_V5\MC15A_V5_1779569544.214\MC15A_V5_1779569544.214\eMachineShop.20.519.ipt
- D:\Tesis\Modelo 3D\CAD\Electronicos\MC15A_V5\MC15A_V5_1779569544.214\MC15A_V5_1779569544.214\eMachineShop.20.520.ipt
- D:\Tesis\Modelo 3D\CAD\Electronicos\MC15A_V5\MC15A_V5_1779569544.214\MC15A_V5_1779569544.214\eMachineShop.20.521.ipt
- D:\Tesis\Modelo 3D\CAD\Electronicos\MC15A_V5\MC15A_V5_1779569544.214\MC15A_V5_1779569544.214\eMachineShop.20.522.ipt
- D:\Tesis\Modelo 3D\CAD\Electronicos\MC15A_V5\MC15A_V5_1779569544.214\MC15A_V5_1779569544.214\eMachineShop.20.523.ipt
- D:\Tesis\Modelo 3D\CAD\Electronicos\MC15A_V5\MC15A_V5_1779569544.214\MC15A_V5_1779569544.214\eMachineShop.20.524.ipt
- D:\Tesis\Modelo 3D\CAD\Electronicos\MC15A_V5\MC15A_V5_1779569544.214\MC15A_V5_1779569544.214\eMachineShop.20.525.ipt
- D:\Tesis\Modelo 3D\CAD\Electronicos\MC15A_V5\MC15A_V5_1779569544.214\MC15A_V5_1779569544.214\eMachineShop.20.526.ipt
- D:\Tesis\Modelo 3D\CAD\Electronicos\MC15A_V5\MC15A_V5_1779569544.214\MC15A_V5_1779569544.214\eMachineShop.20.527.ipt
- D:\Tesis\Modelo 3D\CAD\Electronicos\MC15A_V5\MC15A_V5_1779569544.214\MC15A_V5_1779569544.214\eMachineShop.20.528.ipt
- D:\Tesis\Modelo 3D\CAD\Electronicos\MC15A_V5\MC15A_V5_1779569544.214\MC15A_V5_1779569544.214\eMachineShop.20.529.ipt
- D:\Tesis\Modelo 3D\CAD\Electronicos\MC15A_V5\MC15A_V5_1779569544.214\MC15A_V5_1779569544.214\eMachineShop.20.530.ipt
- D:\Tesis\Modelo 3D\CAD\Electronicos\MC15A_V5\MC15A_V5_1779569544.214\MC15A_V5_1779569544.214\eMachineShop.20.531.ipt
- D:\Tesis\Modelo 3D\CAD\Electronicos\MC15A_V5\MC15A_V5_1779569544.214\MC15A_V5_1779569544.214\eMachineShop.20.532.ipt
- D:\Tesis\Modelo 3D\CAD\Electronicos\MC15A_V5\MC15A_V5_1779569544.214\MC15A_V5_1779569544.214\eMachineShop.20.533.ipt
- D:\Tesis\Modelo 3D\CAD\Electronicos\MC15A_V5\MC15A_V5_1779569544.214\MC15A_V5_1779569544.214\eMachineShop.20.534.ipt
- D:\Tesis\Modelo 3D\CAD\Electronicos\MC15A_V5\MC15A_V5_1779569544.214\MC15A_V5_1779569544.214\eMachineShop.20.535.ipt
- D:\Tesis\Modelo 3D\CAD\Electronicos\MC15A_V5\MC15A_V5_1779569544.214\MC15A_V5_1779569544.214\eMachineShop.20.536.ipt
- D:\Tesis\Modelo 3D\CAD\Electronicos\MC15A_V5\MC15A_V5_1779569544.214\MC15A_V5_1779569544.214\eMachineShop.20.537.ipt
- D:\Tesis\Modelo 3D\CAD\Electronicos\MC15A_V5\MC15A_V5_1779569544.214\MC15A_V5_1779569544.214\eMachineShop.20.538.ipt
- D:\Tesis\Modelo 3D\CAD\Electronicos\MC15A_V5\MC15A_V5_1779569544.214\MC15A_V5_1779569544.214\eMachineShop.20.539.ipt
- D:\Tesis\Modelo 3D\CAD\Electronicos\MC15A_V5\MC15A_V5_1779569544.214\MC15A_V5_1779569544.214\eMachineShop.20.540.ipt
- D:\Tesis\Modelo 3D\CAD\Electronicos\MC15A_V5\MC15A_V5_1779569544.214\MC15A_V5_1779569544.214\eMachineShop.20.541.ipt
- D:\Tesis\Modelo 3D\CAD\Electronicos\MC15A_V5\MC15A_V5_1779569544.214\MC15A_V5_1779569544.214\eMachineShop.20.542.ipt
- D:\Tesis\Modelo 3D\CAD\Electronicos\MC15A_V5\MC15A_V5_1779569544.214\MC15A_V5_1779569544.214\eMachineShop.20.543.ipt
- D:\Tesis\Modelo 3D\CAD\Electronicos\MC15A_V5\MC15A_V5_1779569544.214\MC15A_V5_1779569544.214\eMachineShop.20.544.ipt
- D:\Tesis\Modelo 3D\CAD\Electronicos\MC15A_V5\MC15A_V5_1779569544.214\MC15A_V5_1779569544.214\eMachineShop.20.545.ipt
- D:\Tesis\Modelo 3D\CAD\Electronicos\MC15A_V5\MC15A_V5_1779569544.214\MC15A_V5_1779569544.214\eMachineShop.20.546.ipt
- D:\Tesis\Modelo 3D\CAD\Electronicos\MC15A_V5\MC15A_V5_1779569544.214\MC15A_V5_1779569544.214\eMachineShop.20.547.ipt
- D:\Tesis\Modelo 3D\CAD\Electronicos\MC15A_V5\MC15A_V5_1779569544.214\MC15A_V5_1779569544.214\eMachineShop.20.548.ipt
- D:\Tesis\Modelo 3D\CAD\Electronicos\MC15A_V5\MC15A_V5_1779569544.214\MC15A_V5_1779569544.214\eMachineShop.20.549.ipt
- D:\Tesis\Modelo 3D\CAD\Electronicos\MC15A_V5\MC15A_V5_1779569544.214\MC15A_V5_1779569544.214\eMachineShop.20.550.ipt
- D:\Tesis\Modelo 3D\CAD\Electronicos\MC15A_V5\MC15A_V5_1779569544.214\MC15A_V5_1779569544.214\eMachineShop.20.551.ipt
- D:\Tesis\Modelo 3D\CAD\Electronicos\MC15A_V5\MC15A_V5_1779569544.214\MC15A_V5_1779569544.214\eMachineShop.20.552.ipt
- D:\Tesis\Modelo 3D\CAD\Electronicos\MC15A_V5\MC15A_V5_1779569544.214\MC15A_V5_1779569544.214\eMachineShop.20.553.ipt
- D:\Tesis\Modelo 3D\CAD\Electronicos\MC15A_V5\MC15A_V5_1779569544.214\MC15A_V5_1779569544.214\eMachineShop.20.554.ipt
- D:\Tesis\Modelo 3D\CAD\Electronicos\MC15A_V5\MC15A_V5_1779569544.214\MC15A_V5_1779569544.214\eMachineShop.20.555.ipt
- D:\Tesis\Modelo 3D\CAD\Electronicos\MC15A_V5\MC15A_V5_1779569544.214\MC15A_V5_1779569544.214\eMachineShop.20.556.ipt
- D:\Tesis\Modelo 3D\CAD\Electronicos\MC15A_V5\MC15A_V5_1779569544.214\MC15A_V5_1779569544.214\eMachineShop.20.557.ipt
- D:\Tesis\Modelo 3D\CAD\Electronicos\MC15A_V5\MC15A_V5_1779569544.214\MC15A_V5_1779569544.214\eMachineShop.20.558.ipt
- D:\Tesis\Modelo 3D\CAD\Electronicos\MC15A_V5\MC15A_V5_1779569544.214\MC15A_V5_1779569544.214\eMachineShop.20.559.ipt
- D:\Tesis\Modelo 3D\CAD\Electronicos\MC15A_V5\MC15A_V5_1779569544.214\MC15A_V5_1779569544.214\eMachineShop.20.560.ipt
- D:\Tesis\Modelo 3D\CAD\Electronicos\MC15A_V5\MC15A_V5_1779569544.214\MC15A_V5_1779569544.214\eMachineShop.20.561.ipt
- D:\Tesis\Modelo 3D\CAD\Electronicos\MC15A_V5\MC15A_V5_1779569544.214\MC15A_V5_1779569544.214\eMachineShop.20.562.ipt
- D:\Tesis\Modelo 3D\CAD\Electronicos\MC15A_V5\MC15A_V5_1779569544.214\MC15A_V5_1779569544.214\eMachineShop.20.563.ipt
- D:\Tesis\Modelo 3D\CAD\Electronicos\MC15A_V5\MC15A_V5_1779569544.214\MC15A_V5_1779569544.214\eMachineShop.20.564.ipt
- D:\Tesis\Modelo 3D\CAD\Electronicos\MC15A_V5\MC15A_V5_1779569544.214\MC15A_V5_1779569544.214\eMachineShop.20.565.ipt
- D:\Tesis\Modelo 3D\CAD\Electronicos\MC15A_V5\MC15A_V5_1779569544.214\MC15A_V5_1779569544.214\eMachineShop.20.566.ipt
- D:\Tesis\Modelo 3D\CAD\Electronicos\MC15A_V5\MC15A_V5_1779569544.214\MC15A_V5_1779569544.214\eMachineShop.20.567.ipt
- D:\Tesis\Modelo 3D\CAD\Electronicos\MC15A_V5\MC15A_V5_1779569544.214\MC15A_V5_1779569544.214\eMachineShop.20.568.ipt
- D:\Tesis\Modelo 3D\CAD\Electronicos\MC15A_V5\MC15A_V5_1779569544.214\MC15A_V5_1779569544.214\eMachineShop.20.569.ipt
- D:\Tesis\Modelo 3D\CAD\Electronicos\MC15A_V5\MC15A_V5_1779569544.214\MC15A_V5_1779569544.214\eMachineShop.20.570.ipt
- D:\Tesis\Modelo 3D\CAD\Electronicos\MC15A_V5\MC15A_V5_1779569544.214\MC15A_V5_1779569544.214\eMachineShop.20.571.ipt
- D:\Tesis\Modelo 3D\CAD\Electronicos\MC15A_V5\MC15A_V5_1779569544.214\MC15A_V5_1779569544.214\eMachineShop.20.572.ipt
- D:\Tesis\Modelo 3D\CAD\Electronicos\MC15A_V5\MC15A_V5_1779569544.214\MC15A_V5_1779569544.214\eMachineShop.20.573.ipt
- D:\Tesis\Modelo 3D\CAD\Electronicos\MC15A_V5\MC15A_V5_1779569544.214\MC15A_V5_1779569544.214\eMachineShop.20.574.ipt
- D:\Tesis\Modelo 3D\CAD\Electronicos\MC15A_V5\MC15A_V5_1779569544.214\MC15A_V5_1779569544.214\eMachineShop.20.575.ipt
- D:\Tesis\Modelo 3D\CAD\Electronicos\MC15A_V5\MC15A_V5_1779569544.214\MC15A_V5_1779569544.214\eMachineShop.20.576.ipt
- D:\Tesis\Modelo 3D\CAD\Electronicos\MC15A_V5\MC15A_V5_1779569544.214\MC15A_V5_1779569544.214\eMachineShop.20.577.ipt
- D:\Tesis\Modelo 3D\CAD\Electronicos\MC15A_V5\MC15A_V5_1779569544.214\MC15A_V5_1779569544.214\eMachineShop.20.578.ipt
- D:\Tesis\Modelo 3D\CAD\Electronicos\MC15A_V5\MC15A_V5_1779569544.214\MC15A_V5_1779569544.214\eMachineShop.20.579.ipt
- D:\Tesis\Modelo 3D\CAD\Electronicos\MC15A_V5\MC15A_V5_1779569544.214\MC15A_V5_1779569544.214\eMachineShop.20.580.ipt
- D:\Tesis\Modelo 3D\CAD\Electronicos\MC15A_V5\MC15A_V5_1779569544.214\MC15A_V5_1779569544.214\eMachineShop.20.581.ipt
- D:\Tesis\Modelo 3D\CAD\Electronicos\MC15A_V5\MC15A_V5_1779569544.214\MC15A_V5_1779569544.214\eMachineShop.20.582.ipt
## Components (582 placed, 582 different names)
1. 1383
2. 1384
3. 1385
4. 1386
5. 1387
6. 1388
7. 1389
8. 1390
9. 1391
10. 1392
11. 1393
12. 1394
13. 1395
14. 1396
15. 1397
16. 1398
17. 1399
18. 1400
19. 1401
20. 1402
21. 1403
22. 1404
23. 1405
24. 1406
25. 1407
26. 1408
27. 1409
28. 1410
29. 1411
30. 1412
31. 1413
32. 1414
33. 1415
34. 1416
35. 1417
36. 1418
37. 1419
38. 1420
39. 1421
40. 1422
41. 1423
42. 1424
43. 1425
44. 1426
45. 1427
46. 1428
47. 1429
48. 1430
49. 1431
50. 1432
51. 1433
52. 1434
53. 1435
54. 1436
55. 1437
56. 1438
57. 1439
58. 1440
59. 1441
60. 1442
61. 1443
62. 1444
63. 1445
64. 1446
65. 1447
66. 1448
67. 1449
68. 1450
69. 1451
70. 1452
71. 1453
72. 1454
73. 1455
74. 1456
75. 1457
76. 1458
77. 1459
78. 1460
79. 1461
80. 1462
81. 1463
82. 1464
83. 1465
84. 1466
85. 1467
86. 1468
87. 1469
88. 1470
89. 1471
90. 1472
91. 1473
92. 1474
93. 1475
94. 1476
95. 1477
96. 1478
97. 1479
98. 1480
99. 1481
100. 1482
101. 1483
102. 1484
103. 1485
104. 1486
105. 1487
106. 1488
107. 1489
108. 1490
109. 1491
110. 1492
111. 1493
112. 1494
113. 1495
114. 1496
115. 1497
116. 1498
117. 1499
118. 1500
119. 1501
120. 1502
121. 1503
122. 1504
123. 1505
124. 1506
125. 1507
126. 1508
127. 1509
128. 1510
129. 1511
130. 1512
131. 1513
132. 1514
133. 1515
134. 1516
135. 1517
136. 1518
137. 1519
138. 1520
139. 1521
140. 1522
141. 1523
142. 1524
143. 1525
144. 1526
145. 1527
146. 1528
147. 1529
148. 1530
149. 1531
150. 1532
151. 1533
152. 1534
153. 1535
154. 1536
155. 1537
156. 1538
157. 1539
158. 1540
159. 1541
160. 1542
161. 1543
162. 1544
163. 1545
164. 1546
165. 1547
166. 1548
167. 1549
168. 1550
169. 1551
170. 1552
171. 1553
172. 1554
173. 1555
174. 1556
175. 1557
176. 1558
177. 1559
178. 1560
179. 1561
180. 1562
181. 1563
182. 1564
183. 1565
184. 1566
185. 1567
186. 1568
187. 1569
188. 1570
189. 1571
190. 1572
191. 1573
192. 1574
193. 1575
194. 1576
195. 1577
196. 1578
197. 1579
198. 1580
199. 1581
200. 1582
201. 1583
202. 1584
203. 1585
204. 1586
205. 1587
206. 1588
207. 1589
208. 1590
209. 1591
210. 1592
211. 1593
212. 1594
213. 1595
214. 1596
215. 1597
216. 1598
217. 1599
218. 1600
219. 1601
220. 1602
221. 1603
222. 1604
223. 1605
224. 1606
225. 1607
226. 1608
227. 1609
228. 1610
229. 1611
230. 1612
231. 1613
232. 1614
233. 1615
234. 1616
235. 1617
236. 1618
237. 1619
238. 1620
239. 1621
240. 1622
241. 1623
242. 1624
243. 1625
244. 1626
245. 1627
246. 1628
247. 1629
248. 1630
249. 1631
250. 1632
251. 1633
252. 1634
253. 1635
254. 1636
255. 1637
256. 1638
257. 1639
258. 1640
259. 1641
260. 1642
261. 1643
262. 1644
263. 1645
264. 1646
265. 1647
266. 1648
267. 1649
268. 1650
269. 1651
270. 1652
271. 1653
272. 1654
273. 1655
274. 1656
275. 1657
276. 1658
277. 1659
278. 1660
279. 1661
280. 1662
281. 1663
282. 1664
283. 1665
284. 1666
285. 1667
286. 1668
287. 1669
288. 1670
289. 1671
290. 1672
291. 1673
292. 1674
293. 1675
294. 1676
295. 1677
296. 1678
297. 1679
298. 1680
299. 1681
300. 1682
301. 1683
302. 1684
303. 1685
304. 1686
305. 1687
306. 1688
307. 1689
308. 1690
309. 1691
310. 1692
311. 1693
312. 1694
313. 1695
314. 1696
315. 1697
316. 1698
317. 1699
318. 1700
319. 1701
320. 1702
321. 1703
322. 1704
323. 1705
324. 1706
325. 1707
326. 1708
327. 1709
328. 1710
329. 1711
330. 1712
331. 1713
332. 1714
333. 1715
334. 1716
335. 1717
336. 1718
337. 1719
338. 1720
339. 1721
340. 1722
341. 1723
342. 1724
343. 1725
344. 1726
345. 1727
346. 1728
347. 1729
348. 1730
349. 1731
350. 1732
351. 1733
352. 1734
353. 1735
354. 1736
355. 1737
356. 1738
357. 1739
358. 1740
359. 1741
360. 1742
361. 1743
362. 1744
363. 1745
364. 1746
365. 1747
366. 1748
367. 1749
368. 1750
369. 1751
370. 1752
371. 1753
372. 1754
373. 1755
374. 1756
375. 1757
376. 1758
377. 1759
378. 1760
379. 1761
380. 1762
381. 1763
382. 1764
383. 1765
384. 1766
385. 1767
386. 1768
387. 1769
388. 1770
389. 1771
390. 1772
391. 1773
392. 1774
393. 1775
394. 1776
395. 1777
396. 1778
397. 1779
398. 1780
399. 1781
400. 1782
401. 1783
402. 1784
403. 1785
404. 1786
405. 1787
406. 1788
407. 1789
408. 1790
409. 1791
410. 1792
411. 1793
412. 1794
413. 1795
414. 1796
415. 1797
416. 1798
417. 1799
418. 1800
419. 1801
420. 1802
421. 1803
422. 1804
423. 1805
424. 1806
425. 1807
426. 1808
427. 1809
428. 1810
429. 1811
430. 1812
431. 1813
432. 1814
433. 1815
434. 1816
435. 1817
436. 1818
437. 1819
438. 1820
439. 1821
440. 1822
441. 1823
442. 1824
443. 1825
444. 1826
445. 1827
446. 1828
447. 1829
448. 1830
449. 1831
450. 1832
451. 1833
452. 1834
453. 1835
454. 1836
455. 1837
456. 1838
457. 1839
458. 1840
459. 1841
460. 1842
461. 1843
462. 1844
463. 1845
464. 1846
465. 1847
466. 1848
467. 1849
468. 1850
469. 1851
470. 1852
471. 1853
472. 1854
473. 1855
474. 1856
475. 1857
476. 1858
477. 1859
478. 1860
479. 1861
480. 1862
481. 1863
482. 1864
483. 1865
484. 1866
485. 1867
486. 1868
487. 1869
488. 1870
489. 1871
490. 1872
491. 1873
492. 1874
493. 1875
494. 1876
495. 1877
496. 1878
497. 1879
498. 1880
499. 1881
500. 1882
501. 1883
502. 1884
503. 1885
504. 1886
505. 1887
506. 1888
507. 1889
508. 1890
509. 1891
510. 1892
511. 1893
512. 1894
513. 1895
514. 1896
515. 1897
516. 1898
517. 1899
518. 1900
519. 1901
520. 1902
521. 1903
522. 1904
523. 1905
524. 1906
525. 1907
526. 1908
527. 1909
528. 1910
529. 1911
530. 1912
531. 1913
532. 1914
533. 1915
534. 1916
535. 1917
536. 1918
537. 1919
538. 1920
539. 1921
540. 1922
541. 1923
542. 1924
543. 1925
544. 1926
545. 1927
546. 1928
547. 1929
548. 1930
549. 1931
550. 1932
551. 1933
552. 1934
553. 1935
554. 1936
555. 1937
556. 1938
557. 1939
558. 1940
559. 1941
560. 1942
561. 1943
562. 1944
563. 1945
564. 1946
565. 1947
566. 1948
567. 1949
568. 1950
569. 1951
570. 1952
571. 1953
572. 1954
573. 1955
574. 1956
575. 1957
576. 1958
577. 1959
578. 1960
579. 1961
580. 1962
581. 1963
582. 1964
